# Autodesk Inventor assembly: BackAxleNuts
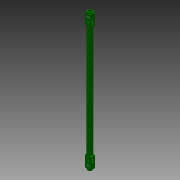
[picture p0: Inventor's stored thumbnail of the model, 180x180]
Saved by Autodesk Inventor 2014 SP1 (Build 180222100, 222)
## iProperties
Created: 2017-01-16
Part Number: BackAxleNuts
Document SubType Name: Assembly
Designer: danielsikar
Author: danielsikar
## Documents named in this file (3)
- C:\Users\danielsikar\Documents\Inventor\IoT-Trike\Assemblies\BackAxleNuts.iam
- C:\Users\danielsikar\Documents\Inventor\IoT-Trike\Parts\Axle270mm.ipt
- C:\Users\danielsikar\Documents\Inventor\Content Center Files\R2014\en-US\BS 3692(1)\BS 3692 - M4(1).ipt
## Components (5 placed, 2 different names)
1. Axle270mm:1 — Mate:1, Mate:2, Mate:3, Mate:4, Mate:5, Mate:6, Mate:7, Mate:8
2. BS 3692 - Metric M4:1 — Mate:1, Mate:2
3. BS 3692 - Metric M4:2 — Mate:5, Mate:6
4. BS 3692 - Metric M4:3 — Mate:3, Mate:4
5. BS 3692 - Metric M4:4 — Mate:7, Mate:8
## Relationships (8: Mate 8)
- Mate:1: Axle270mm:1 ↔ BS 3692 - Metric M4:1
- Mate:2: Axle270mm:1 ↔ BS 3692 - Metric M4:1
- Mate:3: Axle270mm:1 ↔ BS 3692 - Metric M4:3
- Mate:4: Axle270mm:1 ↔ BS 3692 - Metric M4:3
- Mate:5: Axle270mm:1 ↔ BS 3692 - Metric M4:2
- Mate:6: Axle270mm:1 ↔ BS 3692 - Metric M4:2
- Mate:7: Axle270mm:1 ↔ BS 3692 - Metric M4:4
- Mate:8: Axle270mm:1 ↔ BS 3692 - Metric M4:4
